# Autodesk Inventor assembly: servo block assembly
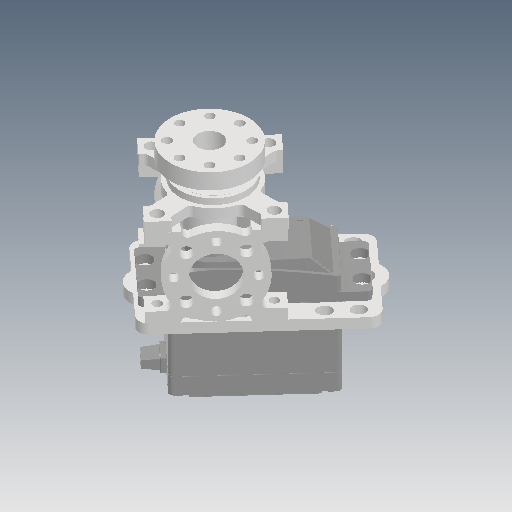
[picture p0: Inventor's stored thumbnail of the model, 512x512]
Saved by Autodesk Inventor 2020 (Build 240168000, 168)
## iProperties
Created: 2019-11-13
Part Number: servo block assembly
Document SubType Name: Assembly
Designer: ball
Author: ball
## Documents named in this file (6)
- C:\FTC\FTC8863CAD\2019 Robot\Collection\servo block assembly.iam
- C:\FTC\FTC8863CAD\Actobotics\637 parts\637110\525122.ipt
- C:\FTC\FTC8863CAD\Actobotics\637 parts\637110\535118 assembly.ipt
- C:\FTC\FTC8863CAD\Actobotics\637 parts\637110\545420.ipt
- C:\FTC\FTC8863CAD\Actobotics\637 parts\637110\575112.ipt
- C:\FTC\FTC8863CAD\GoBilda\2000 Parts\2000-0025-0001 part.ipt
## Components (6 placed, 5 different names)
1. 535118 assembly:1 — Mate:5, Mate:6, Mate:7
2. 545420:1 — Mate:2, Mate:4, Mate:6, Mate:11
3. 575112:1 — Mate:1, Mate:2, Mate:3, Mate:4, Mate:10, Mate:11, Mate:12, Mate:13, Mate:14
4. 545420:2 — Mate:1, Mate:3, Mate:5, Mate:7, Mate:10
5. 2000-0025-0001 part:1 — Mate:12, Mate:13, Mate:14, Mate:15, Mate:16
6. 525122:2 — Mate:15, Mate:16
## Relationships (14: Mate 14)
- Mate:1: 575112:1 ↔ 545420:2
- Mate:2: 545420:1 ↔ 575112:1
- Mate:3: 575112:1 ↔ 545420:2
- Mate:4: 545420:1 ↔ 575112:1
- Mate:5: 535118 assembly:1 ↔ 545420:2
- Mate:6: 535118 assembly:1 ↔ 545420:1
- Mate:7: 535118 assembly:1 ↔ 545420:2
- Mate:10: 575112:1 ↔ 545420:2
- Mate:11: 545420:1 ↔ 575112:1
- Mate:12: 575112:1 ↔ 2000-0025-0001 part:1
- Mate:13: 575112:1 ↔ 2000-0025-0001 part:1
- Mate:14: 575112:1 ↔ 2000-0025-0001 part:1
- Mate:15: 2000-0025-0001 part:1 ↔ 525122:2
- Mate:16: 2000-0025-0001 part:1 ↔ 525122:2
